# Autodesk Inventor assembly: SP
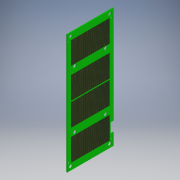
[picture p0: Inventor's stored thumbnail of the model, 180x180]
Saved by Autodesk Inventor 2022 (Build 260153000, 153)
## iProperties
Created: 2021-09-09
Part Number: SP
Document SubType Name: Assembly
Designer: Bowen O'Steen
Author: Bowen O'Steen
## Documents named in this file (3)
- C:\$WorkingFolder\Engineering Data\MemeSat\Solar Panels\SP-03.iam
- C:\$WorkingFolder\Engineering Data\MemeSat\Solar Panels\SolarPCB.ipt
- C:\$WorkingFolder\Engineering Data\MemeSat\Solar Panels\QJcell.ipt
## Components (5 placed, 2 different names)
1. SolarPCB:1 — Mate:1, Mate:2, Flush:1, Mate:3, Mate:4, Mate:5, Mate:6, Mate:7, Mate:10, Mate:11
2. QJcell:3 — Mate:7, Mate:9, Mate:10
3. QJcell:4 — Mate:6, Mate:8, Mate:11
4. QJcell:1 — Mate:3, Mate:4, Mate:5
5. QJcell:2
## Component patterns: (2 elements, first: QJcell:1)
## Relationships (12: Mate 11, Flush 1)
- Mate:1: SolarPCB:1
- Mate:2: SolarPCB:1
- Flush:1: SolarPCB:1
- Mate:3: SolarPCB:1 ↔ QJcell:1
- Mate:4 (1 mm): SolarPCB:1 ↔ QJcell:1
- Mate:5: SolarPCB:1 ↔ QJcell:1
- Mate:6: SolarPCB:1 ↔ QJcell:4
- Mate:7: SolarPCB:1 ↔ QJcell:3
- Mate:8: QJcell:4
- Mate:9: QJcell:3
- Mate:10 (7 mm): SolarPCB:1 ↔ QJcell:3
- Mate:11 (7 mm): SolarPCB:1 ↔ QJcell:4
